# Autodesk Inventor assembly: projectorPanTiltSystem01
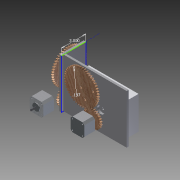
[picture p0: Inventor's stored thumbnail of the model, 180x180]
Saved by Autodesk Inventor 2012 (Build 160160000, 160)
## iProperties
Created: 2014-06-12
Part Number: projectorPanTiltSystem01
Document SubType Name: Assembly
Designer: Byron
Author: Byron
## Documents named in this file (11)
- C:\Documents and Settings\Byron\My Documents\InventorMasterProject\synthesisProjects\projectorPanTilt\projectorPanTiltSystem01.iam
- C:\Documents and Settings\Byron\My Documents\InventorMasterProject\synthesisProjects\projectorPanTilt\aaxaProjector01.ipt
- C:\Documents and Settings\Byron\My Documents\InventorMasterProject\synthesisProjects\projectorPanTilt\projectorPanTiltSystem01\Design Accelerator\Spur Gears1.iam
- C:\Documents and Settings\Byron\My Documents\InventorMasterProject\synthesisProjects\projectorPanTilt\projectorMountingPlate.ipt
- C:\Documents and Settings\Byron\My Documents\InventorMasterProject\synthesisProjects\projectorPanTilt\gearMountSpacer.ipt
- C:\Documents and Settings\Byron\My Documents\InventorMasterProject\synthesisProjects\projectorPanTilt\smallGearBearingBlock.ipt
- C:\Documents and Settings\Byron\My Documents\InventorMasterProject\synthesisProjects\projectorPanTilt\tiltBoxBase.ipt
- C:\Documents and Settings\Byron\My Documents\InventorMasterProject\synthesisProjects\projectorPanTilt\tiltBoxRightSide.ipt
- C:\Documents and Settings\Byron\My Documents\InventorMasterProject\synthesisProjects\projectorPanTilt\projectorPanTiltSystem01\Design Accelerator\Spur Gears2.iam
- C:\Documents and Settings\Byron\My Documents\InventorMasterProject\synthesisProjects\projectorPanTilt\tiltBoxGearSpacerBlock.ipt
- C:\Documents and Settings\Byron\My Documents\InventorMasterProject\synthesisProjects\projectorPanTilt\stepper42BYGH007.ipt
## Components (11 placed, 10 different names)
1. aaxaProjector01:1 — Flush:1
2. Spur Gears:1 [sub-assembly] — Mate:1, Mate:2, Mate:3, Mate:4, Mate:5, Flush:3, Mate:9, Flush:9
3. projectorMountingPlate:1 — Flush:1, Flush:2, Mate:1, Mate:3, Mate:4, Mate:5, Flush:4
4. gearMountSpacer:1 — Flush:2, Mate:2
5. smallGearBearingBlock:1 — Flush:3
6. tiltBoxBase:1 — Flush:4, Flush:5, Mate:6, Flush:6, Flush:7, Angle:1
7. tiltBoxRightSide:1 — Flush:5, Mate:6, Flush:6, Flush:7, Mate:7, Flush:8
8. TiltSpurGears:1 [sub-assembly] — Mate:7, Mate:8
9. tiltBoxGearSpacerBlock:1 — Flush:8, Mate:8
10. stepper42BYGH007:1
11. stepper42BYGH007:2 — Mate:9, Flush:9, Angle:1
## Relationships (19: Flush 9, Mate 9, Angle 1)
- Flush:1: aaxaProjector01:1 ↔ projectorMountingPlate:1
- Flush:2: projectorMountingPlate:1 ↔ gearMountSpacer:1
- Mate:1: Spur Gears:1 ↔ projectorMountingPlate:1
- Mate:2: Spur Gears:1 ↔ gearMountSpacer:1
- Mate:3: Spur Gears:1 ↔ projectorMountingPlate:1
- Mate:4: Spur Gears:1 ↔ projectorMountingPlate:1
- Mate:5: Spur Gears:1 ↔ projectorMountingPlate:1
- Flush:3: Spur Gears:1 ↔ smallGearBearingBlock:1
- Flush:4: projectorMountingPlate:1 ↔ tiltBoxBase:1
- Flush:5: tiltBoxBase:1 ↔ tiltBoxRightSide:1
- Mate:6: tiltBoxBase:1 ↔ tiltBoxRightSide:1
- Flush:6: tiltBoxBase:1 ↔ tiltBoxRightSide:1
- Flush:7 (-6.35 mm): tiltBoxBase:1 ↔ tiltBoxRightSide:1
- Mate:7: tiltBoxRightSide:1 ↔ TiltSpurGears:1
- Flush:8: tiltBoxRightSide:1 ↔ tiltBoxGearSpacerBlock:1
- Mate:8: TiltSpurGears:1 ↔ tiltBoxGearSpacerBlock:1
- Mate:9: Spur Gears:1 ↔ stepper42BYGH007:2
- Flush:9: Spur Gears:1 ↔ stepper42BYGH007:2
- Angle:1 (0 deg): tiltBoxBase:1 ↔ stepper42BYGH007:2
